# Autodesk Inventor assembly: plotter
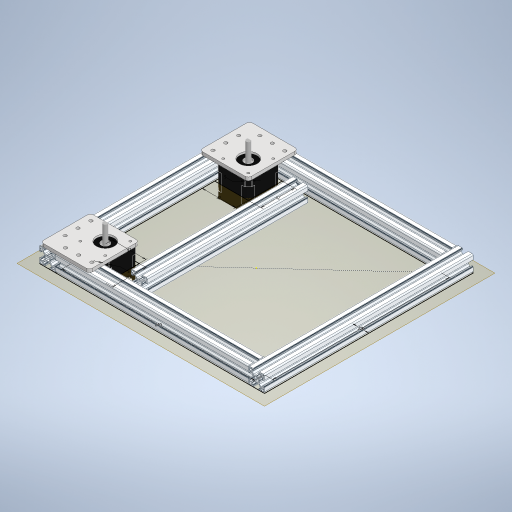
[picture p0: Inventor's stored thumbnail of the model, 512x512]
Saved by Autodesk Inventor 2023.1 (Build 271208000, 208)
## iProperties
Created: 2025-11-24
Part Number: plotter
Document SubType Name: Assembly
Designer: DELL
Author: DELL
## Documents named in this file (8)
- C:\Users\DELL\reposGitHub\VSOSH25-26\models\plotter\plotter.iam
- C:\Users\DELL\reposGitHub\VSOSH25-26\models\plotter\эскиз.ipt
- C:\Users\DELL\reposGitHub\VSOSH25-26\models\import\222LX-Konstruktsionnyy-profil-20kh20L.ipt
- C:\Users\DELL\reposGitHub\VSOSH25-26\models\plotter\профиль2020.ipt
- C:\Users\DELL\reposGitHub\VSOSH25-26\models\import\Schrittmotor-42SHDC3025-24B.ipt
- C:\Users\DELL\reposGitHub\VSOSH25-26\models\plotter\креп_мотора.ipt
- C:\Users\DELL\reposGitHub\VSOSH25-26\models\plotter\креп_мотора_MIR.ipt
- C:\Users\DELL\reposGitHub\VSOSH25-26\models\import\profil.ipt
## Components (10 placed, 9 different names)
1. эскиз:1
2. профиль24Левый — Совмещение:10, Заподлицо:2, Совмещение:12, Заподлицо:3, Совмещение:13, Совмещение:15, Совмещение:16, Совмещение:19, Совмещение:23
3. профиль24правый — Совмещение:1, Заподлицо:1, Совмещение:11, Совмещение:17, Совмещение:18, Совмещение:22
4. профиль16Верх:1 — Заподлицо:1, Совмещение:11, Заподлицо:2, Совмещение:12, Совмещение:15, Совмещение:17, Совмещение:20, Заподлицо:5
5. профиь26низ — Заподлицо:3, Совмещение:13, Совмещение:16, Совмещение:18, Заподлицо:4, Совмещение:21, Совмещение:24
6. Schrittmotor-42SHDC3025-24B:1 — Заподлицо:4, Совмещение:21, Совмещение:22, Заподлицо:6
7. Schrittmotor-42SHDC3025-24B:2 — Заподлицо:5, Совмещение:23, Совмещение:24
8. креп_мотора:1 — Заподлицо:6
9. креп_мотора_MIR:1
10. profil:1 — Совмещение:25
## Relationships (22: Mate 16, Flush 6)
- Совмещение:1 [Mate]: профиль24правый
- Совмещение:10 [Mate]: профиль24Левый
- Заподлицо:1 [Flush]: профиль24правый ↔ профиль16Верх:1
- Совмещение:11 [Mate]: профиль24правый ↔ профиль16Верх:1
- Заподлицо:2 [Flush]: профиль24Левый ↔ профиль16Верх:1
- Совмещение:12 [Mate]: профиль24Левый ↔ профиль16Верх:1
- Заподлицо:3 [Flush]: профиль24Левый ↔ профиь26низ
- Совмещение:13 [Mate]: профиль24Левый ↔ профиь26низ
- Совмещение:15 [Mate]: профиль24Левый ↔ профиль16Верх:1
- Совмещение:16 [Mate]: профиль24Левый ↔ профиь26низ
- Совмещение:17 [Mate]: профиль24правый ↔ профиль16Верх:1
- Совмещение:18 [Mate]: профиль24правый ↔ профиь26низ
- Совмещение:19 [Mate] (110 mm): профиль24Левый
- Совмещение:20 [Mate] (120 mm): профиль16Верх:1
- Заподлицо:4 [Flush]: профиь26низ ↔ Schrittmotor-42SHDC3025-24B:1
- Совмещение:21 [Mate]: профиь26низ ↔ Schrittmotor-42SHDC3025-24B:1
- Совмещение:22 [Mate]: профиль24правый ↔ Schrittmotor-42SHDC3025-24B:1
- Заподлицо:5 [Flush]: профиль16Верх:1 ↔ Schrittmotor-42SHDC3025-24B:2
- Совмещение:23 [Mate]: профиль24Левый ↔ Schrittmotor-42SHDC3025-24B:2
- Совмещение:24 [Mate]: профиь26низ ↔ Schrittmotor-42SHDC3025-24B:2
- Заподлицо:6 [Flush]: Schrittmotor-42SHDC3025-24B:1 ↔ креп_мотора:1
- Совмещение:25 [Mate]: profil:1
